# Autodesk Inventor assembly: Basic Peltier Heat Transfer
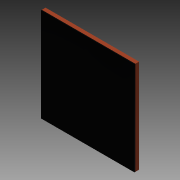
[picture p0: Inventor's stored thumbnail of the model, 180x180]
Saved by Autodesk Inventor 2015 (Build 190159000, 159)
## iProperties
Created: 2015-10-12
Part Number: Basic Peltier Heat Transfer
Document SubType Name: Assembly
Designer: Kyle
Author: Kyle
## Documents named in this file (3)
- C:\Users\Kyle\Documents\Project documentation\Thermoelectric Generator\CAD\Basic Peltier Heat Transfer.iam
- C:\Users\Kyle\Documents\Project documentation\Thermoelectric Generator\CAD\Thermoplastic.ipt
- C:\Users\Kyle\Documents\Project documentation\Thermoelectric Generator\CAD\Copper Plate.ipt
## Components (2 placed, 2 different names)
1. Thermoplastic:1 — Mate:1, Flush:1, Flush:2
2. Copper Plate:1 — Mate:1, Flush:1, Flush:2
## Relationships (3: Flush 2, Mate 1)
- Mate:1: Thermoplastic:1 ↔ Copper Plate:1
- Flush:1: Thermoplastic:1 ↔ Copper Plate:1
- Flush:2: Thermoplastic:1 ↔ Copper Plate:1
